# Autodesk Inventor assembly: krabicka
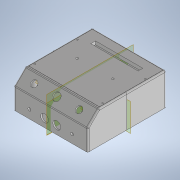
[picture p0: Inventor's stored thumbnail of the model, 180x180]
Saved by Autodesk Inventor 2022 (Build 260153000, 153)
## iProperties
Created: 2022-06-11
Part Number: krabicka
Document SubType Name: Assembly
Designer: adam
Author: adam
## Documents named in this file (3)
- C:\Users\adam\Downloads\krabicka.iam
- C:\Users\adam\Downloads\mavac_vicko.ipt
- C:\Users\adam\Downloads\mavac_krabicka.ipt
## Components (2 placed, 2 different names)
1. mavac_vicko:1 — Mate:1, Mate:2
2. mavac_krabicka:1 — Mate:1, Mate:2, Flush:1
## Relationships (3: Mate 2, Flush 1)
- Mate:1: mavac_vicko:1 ↔ mavac_krabicka:1
- Mate:2: mavac_vicko:1 ↔ mavac_krabicka:1
- Flush:1: mavac_krabicka:1
